# Autodesk Inventor assembly: Drive Assembly
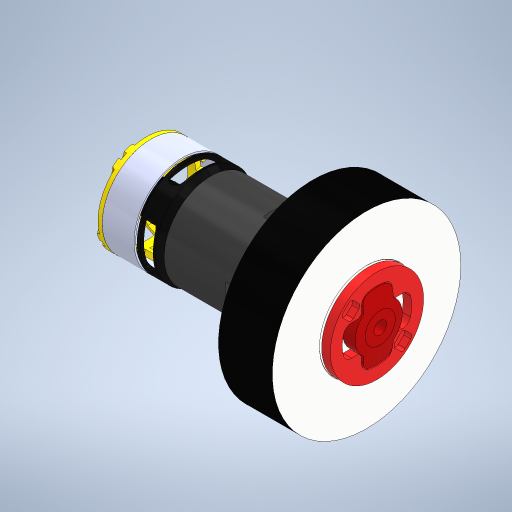
[picture p0: Inventor's stored thumbnail of the model, 512x512]
Saved by Autodesk Inventor 2023.2 (Build 272271000, 271)
## iProperties
Created: 2022-09-11
Part Number: Drive Assembly
Document SubType Name: Assembly
Designer: NCai2
Mass: 12.0236 g
Surface Area: 76.425 cm^2
Volume: 20.9743 cm^3
Density: 0.573256 g/cm^3
Author: NCai2
## Documents named in this file (4)
- E:\Documents\Inventor\Moon Cake V0.13\Drive Assembly.iam
- E:\Documents\Inventor\Moon Cake V0.13\Hubs (Fingertech Twisthub).ipt
- E:\Documents\Inventor\Moon Cake V0.13\Tires (Fingertech Foam Wheels).ipt
- E:\Documents\Inventor\Moon Cake V0.13\RR Brushless\RR-Brushless-Planetary.iam
## Components (3 placed, 3 different names)
1. Hubs (Fingertech Twisthub):1 — Mate:1, Mate:2, Mate:3, Mate:4
2. Tires (Fingertech Foam Wheels):1 — Mate:1, Mate:2
3. RR-Brushless-Planetary:1 [sub-assembly] — Mate:3, Mate:4
## Relationships (4: Mate 4)
- Mate:1: Hubs (Fingertech Twisthub):1 ↔ Tires (Fingertech Foam Wheels):1
- Mate:2: Hubs (Fingertech Twisthub):1 ↔ Tires (Fingertech Foam Wheels):1
- Mate:3: Hubs (Fingertech Twisthub):1 ↔ RR-Brushless-Planetary:1
- Mate:4 (1 mm): Hubs (Fingertech Twisthub):1 ↔ RR-Brushless-Planetary:1
